# Autodesk Inventor assembly: hydraulic_cylinder
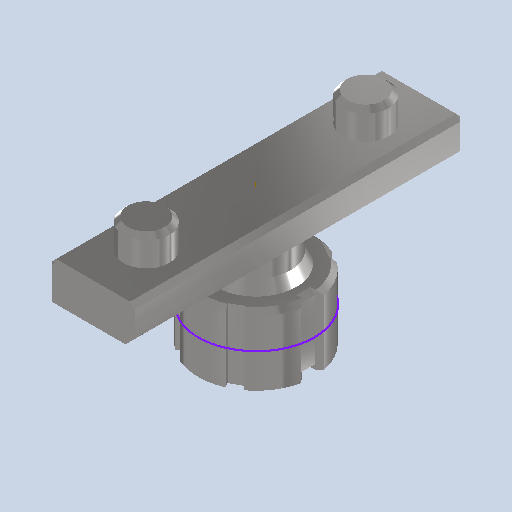
[picture p0: Inventor's stored thumbnail of the model, 512x512]
Saved by Autodesk Inventor 2023 (Build 270158000, 158)
## iProperties
Created: 2023-11-19
Part Number: hydraulic_cylinder
Document SubType Name: Assembly
Designer: Beatrice
Author: Beatrice
## Documents named in this file (3)
- E:\WORKSPACE_2\wheel_changing_assignment\hydraulic_cylinder.iam
- E:\WORKSPACE_2\wheel_changing_assignment\base_hydraulic_pump.ipt
- E:\WORKSPACE_2\wheel_changing_assignment\hydraulic_mech.ipt
## Components (2 placed, 2 different names)
1. base_hydraulic_pump:1 — Insert:1, Mate:1
2. hydraulic_mech:1 — Insert:1, Mate:1
## Relationships (2: Insert 1, Mate 1)
- Insert:1: base_hydraulic_pump:1 ↔ hydraulic_mech:1
- Mate:1: base_hydraulic_pump:1 ↔ hydraulic_mech:1
